# Autodesk Inventor assembly: LED_Strip
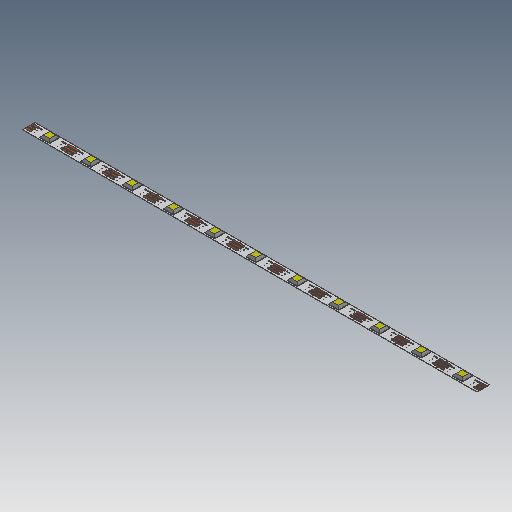
[picture p0: Inventor's stored thumbnail of the model, 512x512]
Saved by Autodesk Inventor 2021.3 (Build 253353000, 353)
## iProperties
Part Number: LED_Strip
Material: Generisch
Document SubType Name: Assembly
Designer: fanki
Mass: 2.29793 g
Surface Area: 82.113 cm^2
Volume: 2.29793 cm^3
Density: 1 g/cm^3
ROT_Weight: 0.002 kg
ROT_Weight_Num: 0.002297931782785665
Author: fanki
## Documents named in this file (2)
- C:\kt\WorkSpace\Uhr\CAD\LED_Strip.iam
- C:\kt\WorkSpace\Uhr\CAD\LED_einzel.ipt
## Components (11 placed, 2 different names)
1. --:31 — Fluchtend:1, Passend:1
2. --:32
3. --:33
4. --:34
5. --:35
6. --:36 — Fluchtend:2
7. --:37
8. --:38
9. LED_einzel:9
10. LED_einzel:10
11. LED_einzel:11
## Component patterns: (11 elements, first: --:31)
## Relationships (3: Flush 2, Mate 1)
- Fluchtend:1 [Flush]: --:31
- Fluchtend:2 [Flush]: --:36
- Passend:1 [Mate]: --:31
